# Autodesk Inventor assembly: Filter
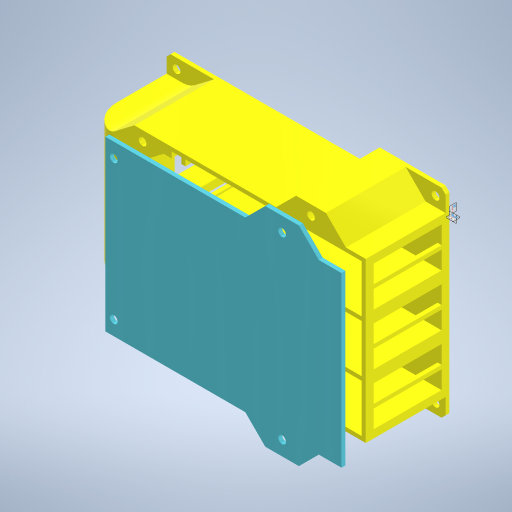
[picture p0: Inventor's stored thumbnail of the model, 512x512]
Saved by Autodesk Inventor 2024.2 (Build 282272000, 272)
## iProperties
Created: 2024-06-02
Part Number: Filter
Document SubType Name: Assembly
Designer: simon
Author: simon
## Documents named in this file (3)
- C:\Users\simon\Documents\Repositories\GrowBox\GrowCarbonFilter\Filter.iam
- C:\Users\simon\Documents\Repositories\GrowBox\GrowCarbonFilter\MainBody.ipt
- C:\Users\simon\Documents\Repositories\GrowBox\GrowCarbonFilter\Cover.ipt
## Components (2 placed, 2 different names)
1. MainBody:1 — Mate:1, Mate:2, Flush:1
2. Cover:1
## Relationships (3: Mate 2, Flush 1)
- Mate:1: MainBody:1
- Mate:2: MainBody:1
- Flush:1: MainBody:1
